# Autodesk Inventor assembly: Motor_Section_Regular_Spacer_MIR1
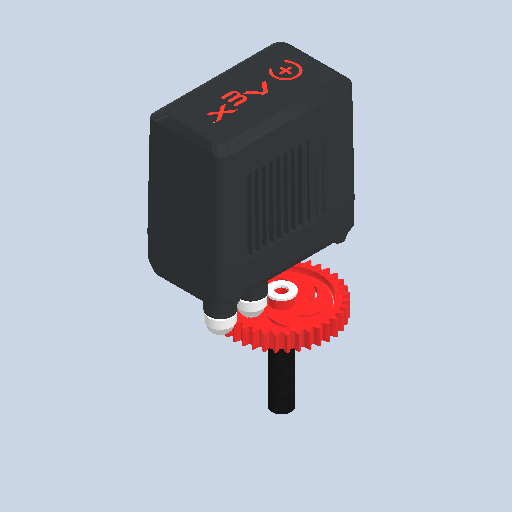
[picture p0: Inventor's stored thumbnail of the model, 512x512]
Saved by Autodesk Inventor 2025.2 (Build 292293000, 293)
## iProperties
Created: 2024-12-08
Part Number: Motor_Section_Regular_Spacer_MIR1
Document SubType Name: Assembly
Designer: joshi
Author: Aditya Koduri
## Documents named in this file (11)
- C:\Users\joshi\Desktop\3388K CAD\Motor_Section_Regular_Spacer_MIR1.iam
- C:\Users\joshi\Desktop\3388K CAD\VEX Main\Motion\Spacers\Washer Teflon\TWasher .375 OD x .03125.ipt
- C:\Users\joshi\Desktop\3388K CAD\VEX Main\Motion\Spacers\Washer Teflon.ipt
- C:\Users\joshi\Desktop\3388K CAD\VEX Main\Motion\Gears\LS 36T Gear_MIR1.ipt
- C:\Users\joshi\Desktop\3388K CAD\VEX Main\Electronics\V5 Motor_MIR1.ipt
- C:\Users\joshi\Desktop\3388K CAD\VEX Main\Motion\Spacers\Spacer Nylon .313 OD\NSpacer .313 OD x .125.ipt
- C:\Users\joshi\Desktop\3388K CAD\VEX Main\Motion\Spacers\Spacer Nylon .313 OD.ipt
- C:\Users\joshi\Desktop\3388K CAD\VEX Main\Structure\Hardware\Screw Steel - Hex\SScrew Hex Smooth .500.ipt
- C:\Users\joshi\Desktop\3388K CAD\VEX Main\Structure\Hardware\Screw Steel - Hex.ipt
- C:\Users\joshi\Desktop\3388K CAD\VEX Main\Motion\Spacers\Spacer Plastic\PSpacer 8.0.ipt
- C:\Users\joshi\Desktop\3388K CAD\VEX Main\Motion\Spacers\Spacer Plastic.ipt
## Components (11 placed, 6 different names)
1. TWasher .375 OD x .03125:1 — Insert:1
2. LS 36T Gear_MIR1:1 — Insert:1, Insert:11
3. V5 Motor_MIR1:1 — Insert:6, Insert:7
4. NSpacer .313 OD x .125:1 — Insert:6
5. NSpacer .313 OD x .125:2 — Insert:7
6. SScrew Hex Smooth .500:1
7. SScrew Hex Smooth .500:2
8. PSpacer 8.0:1 — Insert:8, Insert:9
9. PSpacer 8.0:2 — Insert:8, Insert:10
10. PSpacer 8.0:3 — Insert:11, Insert:9
11. PSpacer 8.0:4 — Insert:10
## Relationships (7: Insert 7)
- Insert:1: TWasher .375 OD x .03125:1 ↔ LS 36T Gear_MIR1:1
- Insert:6: V5 Motor_MIR1:1 ↔ NSpacer .313 OD x .125:1
- Insert:7: V5 Motor_MIR1:1 ↔ NSpacer .313 OD x .125:2
- Insert:8: PSpacer 8.0:1 ↔ PSpacer 8.0:2
- Insert:11: LS 36T Gear_MIR1:1 ↔ PSpacer 8.0:3
- Insert:9: PSpacer 8.0:1 ↔ PSpacer 8.0:3
- Insert:10: PSpacer 8.0:2 ↔ PSpacer 8.0:4
